# Autodesk Inventor assembly: bed_acrylic_assembly
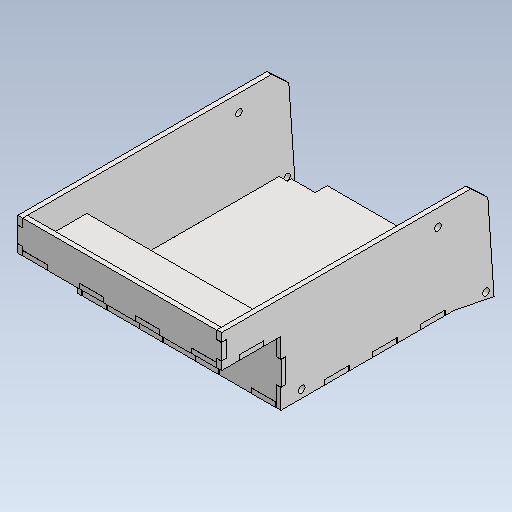
[picture p0: Inventor's stored thumbnail of the model, 512x512]
Saved by Autodesk Inventor 2025 (Build 290162000, 162)
## iProperties
Created: 2025-08-24
Part Number: bed_acrylic_assembly
Document SubType Name: Assembly
Designer: HP
Author: HP
## Documents named in this file (6)
- C:\Users\HP\Documents\GitHub\robotics-dojo-2025\CAD\bed_acrylic_assembly.iam
- C:\Users\HP\Documents\GitHub\robotics-dojo-2025\CAD\bed_acrylic_floor.ipt
- C:\Users\HP\Documents\GitHub\robotics-dojo-2025\CAD\bed_acrylic_side.ipt
- C:\Users\HP\Documents\GitHub\robotics-dojo-2025\CAD\bed_acrylic_lower_front.ipt
- C:\Users\HP\Documents\GitHub\robotics-dojo-2025\CAD\bed_acrylic_upper_floor.ipt
- C:\Users\HP\Documents\GitHub\robotics-dojo-2025\CAD\bed_acrylic_upper_front.ipt
## Components (6 placed, 5 different names)
1. bed_acrylic_floor:1 — Mate:1, Mate:2, Mate:3, Mate:4, Mate:5, Mate:6, Mate:8, Mate:9, Flush:1
2. bed_acrylic_side:1 — Mate:4, Mate:5, Mate:6, Mate:10, Mate:13, Mate:18
3. bed_acrylic_side:2 — Mate:1, Mate:2, Mate:3, Mate:14, Mate:19, Mate:20
4. bed_acrylic_lower_front:1 — Mate:8, Mate:9, Mate:10
5. bed_acrylic_upper_floor:1 — Mate:13, Mate:14, Mate:16, Mate:19
6. bed_acrylic_upper_front:1 — Mate:16, Mate:18, Mate:20
## Relationships (16: Mate 15, Flush 1)
- Mate:1: bed_acrylic_floor:1 ↔ bed_acrylic_side:2
- Mate:2: bed_acrylic_floor:1 ↔ bed_acrylic_side:2
- Mate:3: bed_acrylic_floor:1 ↔ bed_acrylic_side:2
- Mate:4: bed_acrylic_floor:1 ↔ bed_acrylic_side:1
- Mate:5: bed_acrylic_floor:1 ↔ bed_acrylic_side:1
- Mate:6: bed_acrylic_floor:1 ↔ bed_acrylic_side:1
- Mate:8: bed_acrylic_floor:1 ↔ bed_acrylic_lower_front:1
- Mate:9: bed_acrylic_floor:1 ↔ bed_acrylic_lower_front:1
- Mate:10: bed_acrylic_side:1 ↔ bed_acrylic_lower_front:1
- Mate:13: bed_acrylic_side:1 ↔ bed_acrylic_upper_floor:1
- Mate:14: bed_acrylic_side:2 ↔ bed_acrylic_upper_floor:1
- Mate:16: bed_acrylic_upper_floor:1 ↔ bed_acrylic_upper_front:1
- Mate:18: bed_acrylic_side:1 ↔ bed_acrylic_upper_front:1
- Flush:1: bed_acrylic_floor:1
- Mate:19: bed_acrylic_side:2 ↔ bed_acrylic_upper_floor:1
- Mate:20: bed_acrylic_side:2 ↔ bed_acrylic_upper_front:1
